# Autodesk Inventor assembly: Soyuz Stage 3 Sustainerr
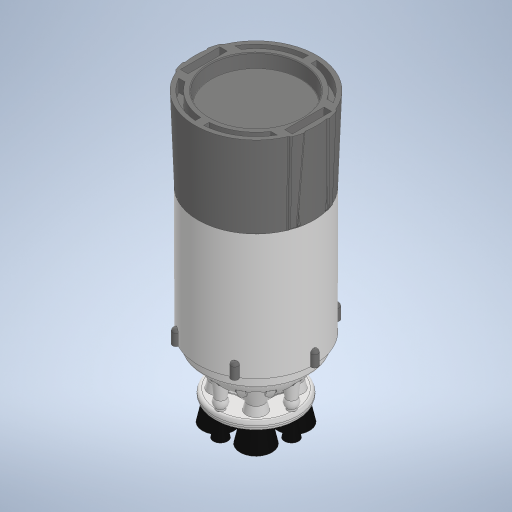
[picture p0: Inventor's stored thumbnail of the model, 512x512]
Saved by Autodesk Inventor 2023 (Build 270158030, 158C)
## iProperties
Created: 2023-01-06
Part Number: Soyuz Stage 3 Sustainerr
Document SubType Name: Assembly
Designer: Imogen Heard
Author: Imogen Heard
## Documents named in this file (3)
- C:\Users\dheard\Documents\Inventor\Inventor_Projects\Soyuz Model\Soyuz Stage 3 Sustainerr.iam
- C:\Users\dheard\Documents\Inventor\Inventor_Projects\Soyuz Model\3rd Stage.ipt
- C:\Users\dheard\Documents\Inventor\Inventor_Projects\Soyuz Model\3rd Stage Part B.ipt
## Components (2 placed, 2 different names)
1. 3rd Stage:1 — Insert:1
2. 3rd Stage Part B:1 — Insert:1
## Relationships (1: Insert 1)
- Insert:1: 3rd Stage:1 ↔ 3rd Stage Part B:1
